# Autodesk Inventor assembly: Kracken with Cover and Boards
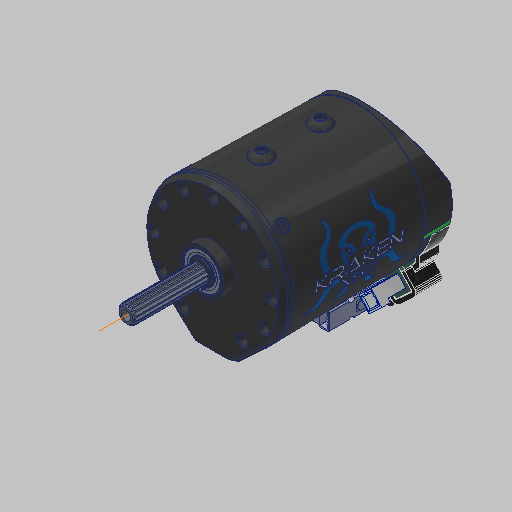
[picture p0: Inventor's stored thumbnail of the model, 512x512]
Saved by Autodesk Inventor 2023.5 (Build 275446000, 446)
## iProperties
Created: 2024-02-20
Part Number: Kracken with Cover and Boards
Document SubType Name: Assembly
Designer: dlangdon
Mass: 555.695 g
Surface Area: 467.249 cm^2
Volume: 211.506 cm^3
Density: 2.62733 g/cm^3
Author: dlangdon
## Documents named in this file (5)
- C:\Users\slick\OneDrive\Desktop\2025-ReefScape---CAD\COMMON PARTS\MOTORS\Kracken with Cover and Boards.iam
- C:\Users\slick\OneDrive\Desktop\2025-ReefScape---CAD\COMMON PARTS\MOTORS\Kracken X60WCP-0940 (1).ipt
- C:\Users\slick\OneDrive\Desktop\2025-ReefScape---CAD\COMMON PARTS\MOTORS\Kracken\kraken-can-adapter.iam
- C:\Users\slick\OneDrive\Desktop\2025-ReefScape---CAD\COMMON PARTS\MOTORS\Kracken\kraken-power-adapter.iam
- C:\Users\slick\OneDrive\Desktop\2025-ReefScape---CAD\COMMON PARTS\MOTORS\Kracken\KrakenCoverA.ipt
## Components (4 placed, 4 different names)
1. Kracken X60WCP-0940 (1):1 — Insert:1, Mate:1, Mate:2, Mate:3, Mate:4
2. kraken-can-adapter:1 [sub-assembly] — Insert:1, Mate:1
3. kraken-power-adapter:1 [sub-assembly] — Mate:2, Mate:3, Mate:4, Mate:5, Mate:6, Flush:1
4. KrakenCoverA:1 — Mate:5, Mate:6, Flush:1
## Relationships (8: Mate 6, Insert 1, Flush 1)
- Insert:1: Kracken X60WCP-0940 (1):1 ↔ kraken-can-adapter:1
- Mate:1 (0.0508 mm): Kracken X60WCP-0940 (1):1 ↔ kraken-can-adapter:1
- Mate:2: Kracken X60WCP-0940 (1):1 ↔ kraken-power-adapter:1
- Mate:3 (0.0508 mm): Kracken X60WCP-0940 (1):1 ↔ kraken-power-adapter:1
- Mate:4: Kracken X60WCP-0940 (1):1 ↔ kraken-power-adapter:1
- Mate:5: kraken-power-adapter:1 ↔ KrakenCoverA:1
- Mate:6: kraken-power-adapter:1 ↔ KrakenCoverA:1
- Flush:1: kraken-power-adapter:1 ↔ KrakenCoverA:1
